# Autodesk Inventor assembly: 110033226_iam_13_散步橋
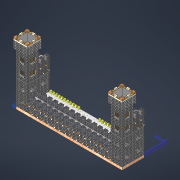
[picture p0: Inventor's stored thumbnail of the model, 180x180]
Saved by Autodesk Inventor 2022 (Build 260153000, 153)
## iProperties
Created: 2022-06-30
Part Number: 110033226_iam_13_散步橋
Document SubType Name: Assembly
Designer: User
Author: User
## Documents named in this file (10)
- D:\D-disk\pomelo\大一\下學期\機械設計製圖\1100332260_LEGOproj_沒有公主城堡\110033226_iam_13_散步橋.iam
- D:\D-disk\pomelo\大一\下學期\機械設計製圖\1100332260_LEGOproj_沒有公主城堡\110033226_ipt_51_散步橋基座.ipt
- D:\D-disk\pomelo\大一\下學期\機械設計製圖\1100332260_LEGOproj_沒有公主城堡\110033226_ipt_28_城堡四圓塔.ipt
- D:\D-disk\pomelo\大一\下學期\機械設計製圖\1100332260_LEGOproj_沒有公主城堡\110033226_iam_06_城堡四角塔.iam
- D:\D-disk\pomelo\大一\下學期\機械設計製圖\1100332260_LEGOproj_沒有公主城堡\110033226_ipt_34_中心城堡圍牆.ipt
- D:\D-disk\pomelo\大一\下學期\機械設計製圖\1100332260_LEGOproj_沒有公主城堡\110033226_ipt_52_散步橋基座二.ipt
- D:\D-disk\pomelo\大一\下學期\機械設計製圖\1100332260_LEGOproj_沒有公主城堡\110033226_ipt_53_散步橋圓柱.ipt
- D:\D-disk\pomelo\大一\下學期\機械設計製圖\1100332260_LEGOproj_沒有公主城堡\110033226_ipt_21_柵欄.ipt
- D:\D-disk\pomelo\大一\下學期\機械設計製圖\1100332260_LEGOproj_沒有公主城堡\110033226_ipt_04_小河.ipt
- D:\D-disk\pomelo\大一\下學期\機械設計製圖\1100332260_LEGOproj_沒有公主城堡\110033226_ipt_37_小河方塊.ipt
## Components (243 placed, 9 different names)
1. 110033226_ipt_51_散步橋基座:1 — 貼合:1, 貼合:2, 貼合:3, 貼合:4, 貼合:5, 貼合:6, 貼合:17, 貼合:18, 貼合:19, 貼合:20, 貼合:21, 貼合:22, 貼合:23, 貼合:24, 貼合:25, 貼合:26, 貼合:27, 貼合:28, 貼合:30, 貼合:35, 齊平:1, 貼合:36, 貼合:37, 貼合:38, 貼合:39
2. 110033226_ipt_52_散步橋基座二:1 — 貼合:23, 貼合:24, 貼合:25, 貼合:29, 貼合:31, 貼合:32, 貼合:33
3. 110033226_ipt_21_柵欄:23 — 貼合:32, 貼合:33, 貼合:34
4. 110033226_iam_06_城堡四角塔:1 [sub-assembly] — 貼合:7, 貼合:8, 貼合:9
5. 110033226_iam_06_城堡四角塔:2 [sub-assembly]
6. 110033226_ipt_34_中心城堡圍牆:9 — 貼合:17, 貼合:18, 貼合:19
7. 110033226_ipt_34_中心城堡圍牆:10
8. 110033226_ipt_34_中心城堡圍牆:11
9. 110033226_ipt_34_中心城堡圍牆:12
10. 110033226_ipt_34_中心城堡圍牆:13
11. 110033226_ipt_34_中心城堡圍牆:14
12. 110033226_ipt_34_中心城堡圍牆:15
13. 110033226_ipt_34_中心城堡圍牆:16
14. 110033226_ipt_34_中心城堡圍牆:17
15. 110033226_ipt_34_中心城堡圍牆:18
16. 110033226_ipt_34_中心城堡圍牆:19
17. 110033226_ipt_34_中心城堡圍牆:20
18. 110033226_ipt_34_中心城堡圍牆:21
19. 110033226_ipt_34_中心城堡圍牆:22
20. 110033226_ipt_34_中心城堡圍牆:23
21. 110033226_ipt_34_中心城堡圍牆:24 — 貼合:20, 貼合:21, 貼合:22
22. 110033226_ipt_34_中心城堡圍牆:25
23. 110033226_ipt_34_中心城堡圍牆:26
24. 110033226_ipt_34_中心城堡圍牆:27
25. 110033226_ipt_34_中心城堡圍牆:28
26. 110033226_ipt_34_中心城堡圍牆:29
27. 110033226_ipt_34_中心城堡圍牆:30
28. 110033226_ipt_34_中心城堡圍牆:31
29. 110033226_ipt_34_中心城堡圍牆:32
30. 110033226_ipt_34_中心城堡圍牆:33
31. 110033226_ipt_34_中心城堡圍牆:34
32. 110033226_ipt_34_中心城堡圍牆:35
33. 110033226_ipt_34_中心城堡圍牆:36
34. 110033226_ipt_34_中心城堡圍牆:37
35. 110033226_ipt_34_中心城堡圍牆:38
36. 110033226_ipt_53_散步橋圓柱:1 — 貼合:26, 貼合:27, 貼合:28
37. 110033226_ipt_53_散步橋圓柱:4
38. 110033226_ipt_53_散步橋圓柱:5
39. 110033226_ipt_53_散步橋圓柱:6
40. 110033226_ipt_53_散步橋圓柱:7
41. 110033226_ipt_53_散步橋圓柱:8
42. 110033226_ipt_53_散步橋圓柱:9
43. 110033226_ipt_53_散步橋圓柱:10
44. 110033226_ipt_53_散步橋圓柱:11
45. 110033226_ipt_53_散步橋圓柱:12
46. 110033226_ipt_53_散步橋圓柱:13
47. 110033226_ipt_53_散步橋圓柱:14
48. 110033226_ipt_53_散步橋圓柱:15
49. 110033226_ipt_53_散步橋圓柱:16
50. 110033226_ipt_53_散步橋圓柱:17
51. 110033226_ipt_53_散步橋圓柱:18
52. 110033226_ipt_53_散步橋圓柱:19
53. 110033226_ipt_53_散步橋圓柱:20
54. 110033226_ipt_53_散步橋圓柱:21
55. 110033226_ipt_53_散步橋圓柱:22
56. 110033226_ipt_53_散步橋圓柱:23
57. 110033226_ipt_53_散步橋圓柱:24
58. 110033226_ipt_53_散步橋圓柱:25
59. 110033226_ipt_53_散步橋圓柱:26
60. 110033226_ipt_04_小河:1 — 貼合:35, 齊平:1, 貼合:36
61. 110033226_ipt_04_小河:2
62. 110033226_ipt_04_小河:3
63. 110033226_ipt_04_小河:4
64. 110033226_ipt_04_小河:5
65. 110033226_ipt_04_小河:6
66. 110033226_ipt_04_小河:7
67. 110033226_ipt_04_小河:8
68. 110033226_ipt_04_小河:9
69. 110033226_ipt_04_小河:10
70. 110033226_ipt_04_小河:11
71. 110033226_ipt_04_小河:12
72. 110033226_ipt_04_小河:13
73. 110033226_ipt_04_小河:14
74. 110033226_ipt_04_小河:15
75. 110033226_ipt_04_小河:16
76. 110033226_ipt_04_小河:17
77. 110033226_ipt_04_小河:18
78. 110033226_ipt_04_小河:19
79. 110033226_ipt_04_小河:20
80. 110033226_ipt_04_小河:21
81. 110033226_ipt_04_小河:22
82. 110033226_ipt_04_小河:23
83. 110033226_ipt_04_小河:24
84. 110033226_ipt_37_小河方塊:1 — 貼合:37, 貼合:38, 貼合:39
85. 110033226_ipt_37_小河方塊:2
86. 110033226_ipt_37_小河方塊:3
87. 110033226_ipt_37_小河方塊:4
88. 110033226_ipt_37_小河方塊:5
89. 110033226_ipt_37_小河方塊:6
90. 110033226_ipt_37_小河方塊:7
91. 110033226_ipt_37_小河方塊:8
92. 110033226_ipt_37_小河方塊:9
93. 110033226_ipt_37_小河方塊:10
94. 110033226_ipt_37_小河方塊:11
95. 110033226_ipt_37_小河方塊:12
96. 110033226_ipt_37_小河方塊:13
97. 110033226_ipt_37_小河方塊:14
98. 110033226_ipt_37_小河方塊:15
99. 110033226_ipt_37_小河方塊:16
100. 110033226_ipt_37_小河方塊:17
101. 110033226_ipt_37_小河方塊:18
102. 110033226_ipt_37_小河方塊:19
103. 110033226_ipt_37_小河方塊:20
104. 110033226_ipt_37_小河方塊:21
105. 110033226_ipt_37_小河方塊:22
106. 110033226_ipt_37_小河方塊:23
107. 110033226_ipt_37_小河方塊:24
108. 110033226_ipt_37_小河方塊:25
109. 110033226_ipt_37_小河方塊:26
110. 110033226_ipt_37_小河方塊:27
111. 110033226_ipt_37_小河方塊:28
112. 110033226_ipt_37_小河方塊:29
113. 110033226_ipt_37_小河方塊:30
114. 110033226_ipt_37_小河方塊:31
115. 110033226_ipt_37_小河方塊:32
116. 110033226_ipt_37_小河方塊:33
117. 110033226_ipt_37_小河方塊:34
118. 110033226_ipt_37_小河方塊:35
119. 110033226_ipt_37_小河方塊:36
120. 110033226_ipt_37_小河方塊:37
121. 110033226_ipt_37_小河方塊:38
122. 110033226_ipt_37_小河方塊:39
123. 110033226_ipt_37_小河方塊:40
124. 110033226_ipt_37_小河方塊:41
125. 110033226_ipt_37_小河方塊:42
126. 110033226_ipt_37_小河方塊:43
127. 110033226_ipt_37_小河方塊:44
128. 110033226_ipt_37_小河方塊:45
129. 110033226_ipt_37_小河方塊:46
130. 110033226_ipt_37_小河方塊:47
131. 110033226_ipt_37_小河方塊:48
132. 110033226_ipt_37_小河方塊:49
133. 110033226_ipt_37_小河方塊:50
134. 110033226_ipt_37_小河方塊:51
135. 110033226_ipt_37_小河方塊:52
136. 110033226_ipt_37_小河方塊:53
137. 110033226_ipt_37_小河方塊:54
138. 110033226_ipt_37_小河方塊:55
139. 110033226_ipt_37_小河方塊:56
140. 110033226_ipt_37_小河方塊:57
141. 110033226_ipt_37_小河方塊:58
142. 110033226_ipt_37_小河方塊:59
143. 110033226_ipt_37_小河方塊:60
144. 110033226_ipt_37_小河方塊:61
145. 110033226_ipt_37_小河方塊:62
146. 110033226_ipt_37_小河方塊:63
147. 110033226_ipt_37_小河方塊:64
148. 110033226_ipt_37_小河方塊:65
149. 110033226_ipt_37_小河方塊:66
150. 110033226_ipt_37_小河方塊:67
151. 110033226_ipt_37_小河方塊:68
152. 110033226_ipt_37_小河方塊:69
153. 110033226_ipt_37_小河方塊:70
154. 110033226_ipt_37_小河方塊:71
155. 110033226_ipt_37_小河方塊:72
156. 110033226_ipt_37_小河方塊:73
157. 110033226_ipt_37_小河方塊:74
158. 110033226_ipt_37_小河方塊:75
159. 110033226_ipt_37_小河方塊:76
160. 110033226_ipt_37_小河方塊:77
161. 110033226_ipt_37_小河方塊:78
162. 110033226_ipt_37_小河方塊:79
163. 110033226_ipt_37_小河方塊:80
164. 110033226_ipt_37_小河方塊:81
165. 110033226_ipt_37_小河方塊:82
166. 110033226_ipt_37_小河方塊:83
167. 110033226_ipt_37_小河方塊:84
168. 110033226_ipt_37_小河方塊:85
169. 110033226_ipt_37_小河方塊:86
170. 110033226_ipt_37_小河方塊:87
171. 110033226_ipt_37_小河方塊:88
172. 110033226_ipt_37_小河方塊:89
173. 110033226_ipt_37_小河方塊:90
174. 110033226_ipt_37_小河方塊:91 — 貼合:42
175. 110033226_ipt_37_小河方塊:92
176. 110033226_ipt_37_小河方塊:93
177. 110033226_ipt_37_小河方塊:94
178. 110033226_ipt_37_小河方塊:95
179. 110033226_ipt_37_小河方塊:96
180. 110033226_ipt_37_小河方塊:97 — 貼合:40, 貼合:41
181. 110033226_ipt_37_小河方塊:98
182. 110033226_ipt_37_小河方塊:99
183. 110033226_ipt_37_小河方塊:100
184. 110033226_ipt_37_小河方塊:101
185. 110033226_ipt_37_小河方塊:102
186. 110033226_ipt_37_小河方塊:103 — 貼合:40, 貼合:41, 貼合:42
187. 110033226_ipt_37_小河方塊:104
188. 110033226_ipt_37_小河方塊:105
189. 110033226_ipt_37_小河方塊:106
190. 110033226_ipt_37_小河方塊:107
191. 110033226_ipt_37_小河方塊:108
192. 110033226_ipt_37_小河方塊:109
193. 110033226_ipt_37_小河方塊:110
194. 110033226_ipt_37_小河方塊:111
195. 110033226_ipt_37_小河方塊:112
196. 110033226_ipt_37_小河方塊:113
197. 110033226_ipt_37_小河方塊:114
198. 110033226_ipt_37_小河方塊:115
199. 110033226_ipt_37_小河方塊:116
200. 110033226_ipt_37_小河方塊:117
201. 110033226_ipt_37_小河方塊:118
202. 110033226_ipt_37_小河方塊:119
203. 110033226_ipt_37_小河方塊:120
204. 110033226_ipt_37_小河方塊:121
205. 110033226_ipt_37_小河方塊:122
206. 110033226_ipt_37_小河方塊:123
207. 110033226_ipt_37_小河方塊:124
208. 110033226_ipt_37_小河方塊:125
209. 110033226_ipt_37_小河方塊:126
210. 110033226_ipt_28_城堡四圓塔:1 — 貼合:4, 貼合:5, 貼合:6, 貼合:7, 貼合:10, 貼合:11, 貼合:12, 貼合:13, 貼合:14, 貼合:15, 貼合:16
211. 110033226_ipt_28_城堡四圓塔:2 — 貼合:8, 貼合:9
212. 110033226_ipt_28_城堡四圓塔:3
213. 110033226_ipt_28_城堡四圓塔:4
214. 110033226_ipt_34_中心城堡圍牆:1 — 貼合:10, 貼合:11, 貼合:12, 貼合:13
215. 110033226_ipt_34_中心城堡圍牆:3
216. 110033226_ipt_34_中心城堡圍牆:2 — 貼合:14, 貼合:15, 貼合:16
217. 110033226_ipt_34_中心城堡圍牆:4
218. 110033226_ipt_34_中心城堡圍牆:5
219. 110033226_ipt_34_中心城堡圍牆:6
220. 110033226_ipt_34_中心城堡圍牆:7
221. 110033226_ipt_34_中心城堡圍牆:8
222. 110033226_ipt_21_柵欄:1 — 貼合:29, 貼合:30, 貼合:31
223. 110033226_ipt_21_柵欄:2
224. 110033226_ipt_21_柵欄:3
225. 110033226_ipt_21_柵欄:4
226. 110033226_ipt_21_柵欄:5
227. 110033226_ipt_21_柵欄:6
228. 110033226_ipt_21_柵欄:7
229. 110033226_ipt_21_柵欄:8
230. 110033226_ipt_21_柵欄:9
231. 110033226_ipt_21_柵欄:10
232. 110033226_ipt_21_柵欄:11
233. 110033226_ipt_21_柵欄:12
234. 110033226_ipt_21_柵欄:13
235. 110033226_ipt_21_柵欄:14
236. 110033226_ipt_21_柵欄:15
237. 110033226_ipt_21_柵欄:16
238. 110033226_ipt_21_柵欄:17
239. 110033226_ipt_21_柵欄:18
240. 110033226_ipt_21_柵欄:19
241. 110033226_ipt_21_柵欄:20
242. 110033226_ipt_21_柵欄:21
243. 110033226_ipt_21_柵欄:22 — 貼合:34
## Component patterns: (2 elements), (2 elements, first: 110033226_iam_06_城堡四角塔:1), (2 elements), (15 elements, first: 110033226_ipt_34_中心城堡圍牆:9), (15 elements, first: 110033226_ipt_34_中心城堡圍牆:24), (24 elements, first: 110033226_ipt_53_散步橋圓柱:1), (2 elements), (24 elements, first: 110033226_ipt_04_小河:1), (102 elements, first: 110033226_ipt_37_小河方塊:1), (24 elements, first: 110033226_ipt_37_小河方塊:103), (2 elements, first: 110033226_ipt_28_城堡四圓塔:1), 元件陣列 1:2 (2 elements), (2 elements, first: 110033226_ipt_34_中心城堡圍牆:1), (2 elements, first: 110033226_ipt_34_中心城堡圍牆:2), 元件陣列 4:2 (2 elements), 元件陣列 5:2 (2 elements), (11 elements, first: 110033226_ipt_21_柵欄:1), 元件陣列 10:2 (11 elements)
## Relationships (43: Mate 42, Flush 1)
- 貼合:1 [Mate]: 110033226_ipt_51_散步橋基座:1
- 貼合:2 [Mate]: 110033226_ipt_51_散步橋基座:1
- 貼合:3 [Mate]: 110033226_ipt_51_散步橋基座:1
- 貼合:4 [Mate]: 110033226_ipt_51_散步橋基座:1 ↔ 110033226_ipt_28_城堡四圓塔:1
- 貼合:5 [Mate]: 110033226_ipt_51_散步橋基座:1 ↔ 110033226_ipt_28_城堡四圓塔:1
- 貼合:6 [Mate]: 110033226_ipt_51_散步橋基座:1 ↔ 110033226_ipt_28_城堡四圓塔:1
- 貼合:7 [Mate]: 110033226_iam_06_城堡四角塔:1 ↔ 110033226_ipt_28_城堡四圓塔:1
- 貼合:8 [Mate]: 110033226_iam_06_城堡四角塔:1 ↔ 110033226_ipt_28_城堡四圓塔:2
- 貼合:9 [Mate]: 110033226_iam_06_城堡四角塔:1 ↔ 110033226_ipt_28_城堡四圓塔:2
- 貼合:10 [Mate]: 110033226_ipt_28_城堡四圓塔:1 ↔ 110033226_ipt_34_中心城堡圍牆:1
- 貼合:11 [Mate]: 110033226_ipt_28_城堡四圓塔:1 ↔ 110033226_ipt_34_中心城堡圍牆:1
- 貼合:12 [Mate]: 110033226_ipt_28_城堡四圓塔:1 ↔ 110033226_ipt_34_中心城堡圍牆:1
- 貼合:13 [Mate]: 110033226_ipt_28_城堡四圓塔:1 ↔ 110033226_ipt_34_中心城堡圍牆:1
- 貼合:14 [Mate]: 110033226_ipt_28_城堡四圓塔:1 ↔ 110033226_ipt_34_中心城堡圍牆:2
- 貼合:15 [Mate]: 110033226_ipt_28_城堡四圓塔:1 ↔ 110033226_ipt_34_中心城堡圍牆:2
- 貼合:16 [Mate]: 110033226_ipt_28_城堡四圓塔:1 ↔ 110033226_ipt_34_中心城堡圍牆:2
- 貼合:17 [Mate]: 110033226_ipt_51_散步橋基座:1 ↔ 110033226_ipt_34_中心城堡圍牆:9
- 貼合:18 [Mate]: 110033226_ipt_51_散步橋基座:1 ↔ 110033226_ipt_34_中心城堡圍牆:9
- 貼合:19 [Mate]: 110033226_ipt_51_散步橋基座:1 ↔ 110033226_ipt_34_中心城堡圍牆:9
- 貼合:20 [Mate]: 110033226_ipt_51_散步橋基座:1 ↔ 110033226_ipt_34_中心城堡圍牆:24
- 貼合:21 [Mate]: 110033226_ipt_51_散步橋基座:1 ↔ 110033226_ipt_34_中心城堡圍牆:24
- 貼合:22 [Mate]: 110033226_ipt_51_散步橋基座:1 ↔ 110033226_ipt_34_中心城堡圍牆:24
- 貼合:23 [Mate] (23.5 mm): 110033226_ipt_51_散步橋基座:1 ↔ 110033226_ipt_52_散步橋基座二:1
- 貼合:24 [Mate]: 110033226_ipt_51_散步橋基座:1 ↔ 110033226_ipt_52_散步橋基座二:1
- 貼合:25 [Mate]: 110033226_ipt_51_散步橋基座:1 ↔ 110033226_ipt_52_散步橋基座二:1
- 貼合:26 [Mate]: 110033226_ipt_51_散步橋基座:1 ↔ 110033226_ipt_53_散步橋圓柱:1
- 貼合:27 [Mate]: 110033226_ipt_51_散步橋基座:1 ↔ 110033226_ipt_53_散步橋圓柱:1
- 貼合:28 [Mate]: 110033226_ipt_51_散步橋基座:1 ↔ 110033226_ipt_53_散步橋圓柱:1
- 貼合:29 [Mate]: 110033226_ipt_52_散步橋基座二:1 ↔ 110033226_ipt_21_柵欄:1
- 貼合:30 [Mate]: 110033226_ipt_51_散步橋基座:1 ↔ 110033226_ipt_21_柵欄:1
- 貼合:31 [Mate]: 110033226_ipt_52_散步橋基座二:1 ↔ 110033226_ipt_21_柵欄:1
- 貼合:32 [Mate]: 110033226_ipt_52_散步橋基座二:1 ↔ 110033226_ipt_21_柵欄:23
- 貼合:33 [Mate]: 110033226_ipt_52_散步橋基座二:1 ↔ 110033226_ipt_21_柵欄:23
- 貼合:34 [Mate]: 110033226_ipt_21_柵欄:23 ↔ 110033226_ipt_21_柵欄:22
- 貼合:35 [Mate]: 110033226_ipt_51_散步橋基座:1 ↔ 110033226_ipt_04_小河:1
- 齊平:1 [Flush]: 110033226_ipt_51_散步橋基座:1 ↔ 110033226_ipt_04_小河:1
- 貼合:36 [Mate]: 110033226_ipt_51_散步橋基座:1 ↔ 110033226_ipt_04_小河:1
- 貼合:37 [Mate]: 110033226_ipt_51_散步橋基座:1 ↔ 110033226_ipt_37_小河方塊:1
- 貼合:38 [Mate]: 110033226_ipt_51_散步橋基座:1 ↔ 110033226_ipt_37_小河方塊:1
- 貼合:39 [Mate]: 110033226_ipt_51_散步橋基座:1 ↔ 110033226_ipt_37_小河方塊:1
- 貼合:40 [Mate]: 110033226_ipt_37_小河方塊:97 ↔ 110033226_ipt_37_小河方塊:103
- 貼合:41 [Mate]: 110033226_ipt_37_小河方塊:97 ↔ 110033226_ipt_37_小河方塊:103
- 貼合:42 [Mate]: 110033226_ipt_37_小河方塊:91 ↔ 110033226_ipt_37_小河方塊:103
